# Autodesk Inventor assembly: HyperCube Evolution
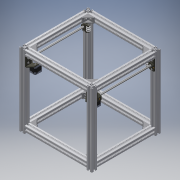
[picture p0: Inventor's stored thumbnail of the model, 180x180]
Saved by Autodesk Inventor 2016 (Build 200138000, 138)
## iProperties
Created: 2017-04-09
Part Number: HyperCube Evolution
Document SubType Name: Assembly
Designer: Scott
Author: Scott
## Documents named in this file (6)
- E:\Scott Projects\3D Printing\CoreXY\HyperCube Evolution.iam
- E:\Scott Projects\3D Printing\CoreXY\HyperCube Evolution frame.iam
- E:\Scott Projects\3D Printing\CoreXY\Y Axis Assembly 1.0.iam
- E:\Scott Projects\3D Printing\CoreXY\Y Axis Assembly 1.0_MIR.iam
- C:\Users\Scott\Documents\Inventor\Content Center Files\R2016\en-US\ANSI B18.3.4M(1)\ANSI B18.3.4M - M5 x 0.8 x 10(2).ipt
- C:\Users\Scott\Documents\Inventor\Content Center Files\R2016\en-US\ANSI B18.3.4M(1)\ANSI B18.3.4M - M6 x 1 x 10(2).ipt
## Components (13 placed, 5 different names)
1. HyperCube Evolution frame:1 [sub-assembly] — Flush:1, Flush:2, Flush:3, Mate:1, Mate:2, Mate:3, Mate:6, Mate:7, Mate:8
2. Y Axis Assembly 1.0:1 [sub-assembly] — Mate:1, Mate:2, Mate:3, Insert:2, Insert:3, Insert:6, Insert:7, Insert:8
3. Y Axis Assembly 1.0_MIR:1 [sub-assembly] — Mate:6, Mate:7, Mate:8, Insert:1, Insert:4, Insert:5, Insert:9, Insert:10
4. Broached Hexagon Socket Button Head Cap Screw - Metric M5 x 0.8 x 10:1 — Insert:1
5. Broached Hexagon Socket Button Head Cap Screw - Metric M5 x 0.8 x 10:2 — Insert:2
6. Broached Hexagon Socket Button Head Cap Screw - Metric M5 x 0.8 x 10:3 — Insert:3
7. Broached Hexagon Socket Button Head Cap Screw - Metric M5 x 0.8 x 10:4 — Insert:4
8. Broached Hexagon Socket Button Head Cap Screw - Metric M6 x 1 x 10:1 — Insert:5
9. Broached Hexagon Socket Button Head Cap Screw - Metric M5 x 0.8 x 10:5 — Insert:6
10. Broached Hexagon Socket Button Head Cap Screw - Metric M5 x 0.8 x 10:6 — Insert:7
11. Broached Hexagon Socket Button Head Cap Screw - Metric M5 x 0.8 x 10:7 — Insert:8
12. Broached Hexagon Socket Button Head Cap Screw - Metric M5 x 0.8 x 10:8 — Insert:9
13. Broached Hexagon Socket Button Head Cap Screw - Metric M5 x 0.8 x 10:9 — Insert:10
## Relationships (19: Insert 10, Mate 6, Flush 3)
- Flush:1: HyperCube Evolution frame:1
- Flush:2: HyperCube Evolution frame:1
- Flush:3: HyperCube Evolution frame:1
- Mate:1: HyperCube Evolution frame:1 ↔ Y Axis Assembly 1.0:1
- Mate:2: HyperCube Evolution frame:1 ↔ Y Axis Assembly 1.0:1
- Mate:3: HyperCube Evolution frame:1 ↔ Y Axis Assembly 1.0:1
- Mate:6: HyperCube Evolution frame:1 ↔ Y Axis Assembly 1.0_MIR:1
- Mate:7: HyperCube Evolution frame:1 ↔ Y Axis Assembly 1.0_MIR:1
- Mate:8: HyperCube Evolution frame:1 ↔ Y Axis Assembly 1.0_MIR:1
- Insert:1: Y Axis Assembly 1.0_MIR:1 ↔ Broached Hexagon Socket Button Head Cap Screw - Metric M5 x 0.8 x 10:1
- Insert:2: Y Axis Assembly 1.0:1 ↔ Broached Hexagon Socket Button Head Cap Screw - Metric M5 x 0.8 x 10:2
- Insert:3: Y Axis Assembly 1.0:1 ↔ Broached Hexagon Socket Button Head Cap Screw - Metric M5 x 0.8 x 10:3
- Insert:4: Y Axis Assembly 1.0_MIR:1 ↔ Broached Hexagon Socket Button Head Cap Screw - Metric M5 x 0.8 x 10:4
- Insert:5: Y Axis Assembly 1.0_MIR:1 ↔ Broached Hexagon Socket Button Head Cap Screw - Metric M6 x 1 x 10:1
- Insert:6: Y Axis Assembly 1.0:1 ↔ Broached Hexagon Socket Button Head Cap Screw - Metric M5 x 0.8 x 10:5
- Insert:7: Y Axis Assembly 1.0:1 ↔ Broached Hexagon Socket Button Head Cap Screw - Metric M5 x 0.8 x 10:6
- Insert:8: Y Axis Assembly 1.0:1 ↔ Broached Hexagon Socket Button Head Cap Screw - Metric M5 x 0.8 x 10:7
- Insert:9: Y Axis Assembly 1.0_MIR:1 ↔ Broached Hexagon Socket Button Head Cap Screw - Metric M5 x 0.8 x 10:8
- Insert:10: Y Axis Assembly 1.0_MIR:1 ↔ Broached Hexagon Socket Button Head Cap Screw - Metric M5 x 0.8 x 10:9
